# Autodesk Inventor assembly: Tank Assembly
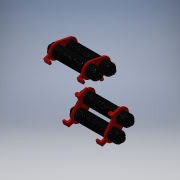
[picture p0: Inventor's stored thumbnail of the model, 180x180]
Saved by Autodesk Inventor 2019.4 (Build 234330000, 330)
## iProperties
Created: 2020-01-30
Part Number: Tank Assembly
Document SubType Name: Assembly
Designer: admin
Author: admin
## Documents named in this file (3)
- C:\Users\Mark\Desktop\7738 Helion Engineering\7738-2020\Robot V2\97995503-9-avt-pp-35\Tank Assembly.iam
- C:\Users\Mark\Desktop\7738 Helion Engineering\7738-2020\Robot V2\97995503-9-avt-pp-35\avt-pp-35.iam
- C:\Users\Mark\Desktop\7738 Helion Engineering\7738-2020\Robot V2\97995503-9-avt-pp-35\Tank Mount.ipt
## Components (8 placed, 2 different names)
1. avt-pp-35:1 [sub-assembly] — Mate:8, Mate:10, Mate:16
2. avt-pp-35:2 [sub-assembly] — Mate:5, Mate:7
3. avt-pp-35:3 [sub-assembly] — Mate:9, Mate:11
4. avt-pp-35:4 [sub-assembly] — Mate:4, Mate:6, Mate:15
5. Tank Mount:1 — Mate:6, Mate:7, Mate:12
6. Tank Mount:2 — Mate:4, Mate:5, Mate:12, Mate:14, Mate:15, Flush:4
7. Tank Mount:3 — Mate:10, Mate:11, Mate:13, Mate:14, Mate:16, Flush:4
8. Tank Mount:4 — Mate:8, Mate:9, Mate:13
## Relationships (20: Mate 16, Flush 4)
- [Mate] (80 mm): avt-pp-35:2 ↔ avt-pp-35:4
- [Flush]: avt-pp-35:2 ↔ avt-pp-35:4
- [Flush]: avt-pp-35:2 ↔ avt-pp-35:3
- [Mate] (80 mm): avt-pp-35:1 ↔ avt-pp-35:3
- [Mate] (80 mm): avt-pp-35:1 ↔ avt-pp-35:3
- [Flush]: avt-pp-35:1 ↔ avt-pp-35:3
- Mate:4: avt-pp-35:4 ↔ Tank Mount:2
- Mate:5: avt-pp-35:2 ↔ Tank Mount:2
- Mate:6: avt-pp-35:4 ↔ Tank Mount:1
- Mate:7: avt-pp-35:2 ↔ Tank Mount:1
- Mate:8: avt-pp-35:1 ↔ Tank Mount:4
- Mate:9: avt-pp-35:3 ↔ Tank Mount:4
- Mate:10: avt-pp-35:1 ↔ Tank Mount:3
- Mate:11: avt-pp-35:3 ↔ Tank Mount:3
- Mate:12 (200 mm): Tank Mount:1 ↔ Tank Mount:2
- Mate:13 (200 mm): Tank Mount:3 ↔ Tank Mount:4
- Mate:14 (238.6 mm): Tank Mount:2 ↔ Tank Mount:3
- Mate:15: avt-pp-35:4 ↔ Tank Mount:2
- Mate:16: avt-pp-35:1 ↔ Tank Mount:3
- Flush:4: Tank Mount:2 ↔ Tank Mount:3
